# Autodesk Inventor assembly: Inner Channel
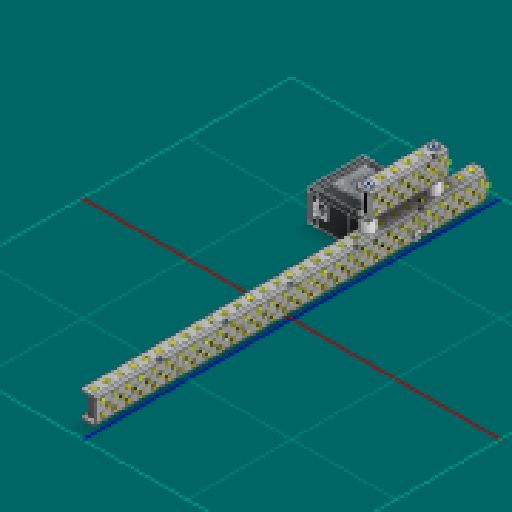
[picture p0: Inventor's stored thumbnail of the model, 512x512]
Saved by Autodesk Inventor 2025 (Build 290162000, 162)
## iProperties
Created: 2024-10-18
Part Number: Inner Channel
Document SubType Name: Assembly
Designer: averey
Author: averey
## Documents named in this file (15)
- C:\Users\avere\VEX\High Stakes\CAD\V2\Chassis\Drivebay Left\Inner Channel.iam
- C:\Users\avere\vex_robotics_high_stakes\hardware\cad\robpros_cad_lib\Structure\C Channel\Aluminum 1x2x1\Alu C 1x2x1x30.ipt
- C:\Users\avere\vex_robotics_high_stakes\hardware\cad\robpros_cad_lib\Structure\C Channel\Aluminum 1x2x1\Alu C 1x2x1x6.ipt
- C:\Users\avere\vex_robotics_high_stakes\hardware\cad\robpros_cad_lib\Motion\Spacers\Spacer Nylon .500 OD\NSpacer White .500 OD x .500.ipt
- C:\Users\avere\vex_robotics_high_stakes\hardware\cad\robpros_cad_lib\Motion\Spacers\Spacer Nylon .500 OD.ipt
- C:\Users\avere\VEX\High Stakes\CAD\ROBOPROS-CAD-Inventor\Motion\Spacers\Spacer Nylon .375 OD\NSpacer .375 OD x .875.ipt
- C:\Users\avere\VEX\High Stakes\CAD\ROBOPROS-CAD-Inventor\Motion\Spacers\Spacer Nylon .375 OD.ipt
- C:\Users\avere\VEX\High Stakes\CAD\ROBOPROS-CAD-Inventor\Structure\Standoff\Standoff .875.ipt
- C:\Users\avere\VEX\High Stakes\CAD\ROBOPROS-CAD-Inventor\Structure\Standoff.ipt
- C:\Users\avere\VEX\High Stakes\CAD\ROBOPROS-CAD-Inventor\Structure\Hardware\Screw Steel - Star\SScrew Star Smooth 1.750.ipt
- C:\Users\avere\VEX\High Stakes\CAD\ROBOPROS-CAD-Inventor\Structure\Hardware\Screw Steel - Star.ipt
- C:\Users\avere\VEX\High Stakes\CAD\ROBOPROS-CAD-Inventor\Structure\Hardware\Screw Steel - Star\SScrew Star Smooth .290.ipt
- C:\Users\avere\VEX\High Stakes\CAD\ROBOPROS-CAD-Inventor\Quick Assemblies\Bearing Flat NScrew Slotted Offset.iam
- C:\Users\avere\VEX\High Stakes\CAD\ROBOPROS-CAD-Inventor\Electronics\V5 Motor.ipt
- C:\Users\avere\VEX\High Stakes\CAD\ROBOPROS-CAD-Inventor\Electronics\V5 Motor (5.5W).ipt
## Components (15 placed, 10 different names)
1. Alu C 1x2x1x30:1 — Mate:1, Insert:7, Mate:2, Insert:8, Insert:9, Insert:10, Mate:3, Insert:11, Mate:4, Insert:12, Mate:5, Insert:13, Mate:6
2. Alu C 1x2x1x6:1 — Insert:6, Insert:14, Mate:7
3. NSpacer White .500 OD x .500:1 — Mate:2
4. NSpacer .375 OD x .875:1
5. Standoff .875:1
6. SScrew Star Smooth 1.750:1 — Insert:8
7. SScrew Star Smooth .290:2
8. SScrew Star Smooth 1.750:3
9. NSpacer White .500 OD x .500:2 — Insert:6, Insert:7
10. Standoff .875:2 — Insert:9
11. Bearing Flat NScrew Slotted Offset:1 [sub-assembly] — Insert:10, Mate:3
12. V5 Motor:1 — Insert:11, Mate:4
13. V5 Motor:2 — Insert:12, Mate:5
14. V5 Motor:3 — Insert:13, Mate:6
15. V5 Motor (5.5W):1 — Insert:14, Mate:7
## Relationships (21: Insert 14, Mate 7)
- Mate:1: Alu C 1x2x1x30:1
- [Insert]: Alu C 1x2x1x6:1 ↔ NSpacer White .500 OD x .500:1
- [Insert]: Alu C 1x2x1x6:1 ↔ NSpacer .375 OD x .875:1
- [Insert]: Alu C 1x2x1x6:1 ↔ Standoff .875:1
- [Insert]: Alu C 1x2x1x6:1 ↔ SScrew Star Smooth .290:2
- [Insert]: Alu C 1x2x1x6:1 ↔ SScrew Star Smooth 1.750:3
- Insert:6: Alu C 1x2x1x6:1 ↔ NSpacer White .500 OD x .500:2
- Insert:7: Alu C 1x2x1x30:1 ↔ NSpacer White .500 OD x .500:2
- Mate:2: Alu C 1x2x1x30:1 ↔ NSpacer White .500 OD x .500:1
- Insert:8: Alu C 1x2x1x30:1 ↔ SScrew Star Smooth 1.750:1
- Insert:9: Alu C 1x2x1x30:1 ↔ Standoff .875:2
- Insert:10: Alu C 1x2x1x30:1 ↔ Bearing Flat NScrew Slotted Offset:1
- Mate:3: Alu C 1x2x1x30:1 ↔ Bearing Flat NScrew Slotted Offset:1
- Insert:11: Alu C 1x2x1x30:1 ↔ V5 Motor:1
- Mate:4: Alu C 1x2x1x30:1 ↔ V5 Motor:1
- Insert:12: Alu C 1x2x1x30:1 ↔ V5 Motor:2
- Mate:5: Alu C 1x2x1x30:1 ↔ V5 Motor:2
- Insert:13: Alu C 1x2x1x30:1 ↔ V5 Motor:3
- Mate:6: Alu C 1x2x1x30:1 ↔ V5 Motor:3
- Insert:14: Alu C 1x2x1x6:1 ↔ V5 Motor (5.5W):1
- Mate:7: Alu C 1x2x1x6:1 ↔ V5 Motor (5.5W):1
## Named parameters: d42_d41 = 0 mm
